# Autodesk Inventor assembly: WheelsWithBearings
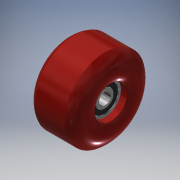
[picture p0: Inventor's stored thumbnail of the model, 180x180]
Saved by Autodesk Inventor 2019 (Build 230136000, 136)
## iProperties
Created: 2020-12-13
Part Number: WheelsWithBearings
Document SubType Name: Assembly
Designer: Anass Hamdi
Author: Anass Hamdi
## Documents named in this file (3)
- C:\Users\Anass Hamdi\OneDrive - Vrije Universiteit Brussel\Documenten\Inventor\Anass Hamdi Project\WheelsWithBearings.iam
- C:\Users\Anass Hamdi\OneDrive - Vrije Universiteit Brussel\Documenten\Inventor\Anass Hamdi Project\Bearings.iam
- C:\Users\Anass Hamdi\OneDrive - Vrije Universiteit Brussel\Documenten\Inventor\Anass Hamdi Project\Wheels 54mm cut.ipt
## Components (3 placed, 2 different names)
1. Bearings:1 [sub-assembly] — Rotational:1
2. Bearings:2 [sub-assembly] — Rotational:2
3. Wheels 54mm cut:1 — Rotational:1, Rotational:2
## Relationships (2: RevoluteJoint 2)
- Rotational:1 [RevoluteJoint]: Bearings:1 ↔ Wheels 54mm cut:1
- Rotational:2 [RevoluteJoint]: Bearings:2 ↔ Wheels 54mm cut:1
